# Autodesk Inventor assembly: placa
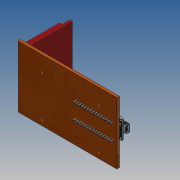
[picture p0: Inventor's stored thumbnail of the model, 180x180]
Saved by Autodesk Inventor 2017 (Build 210142000, 142)
## iProperties
Part Number: placa
Material: Genérico
Document SubType Name: Assembly
Designer: Leo
Author: Leo
## Documents named in this file (5)
- C:\Users\leo.DESKTOP-592E5E6\Dropbox\multiactuador\placa.iam
- C:\Users\leo.DESKTOP-592E5E6\Dropbox\multiactuador\placa\placa circuito.ipt
- C:\Users\leo.DESKTOP-592E5E6\Dropbox\multiactuador\import\arduino nano.ipt
- C:\Users\leo.DESKTOP-592E5E6\Dropbox\multiactuador\componentes\pantalla.ipt
- C:\Users\leo.DESKTOP-592E5E6\Dropbox\multiactuador\componentes\conector mini usb.ipt
## Components (4 placed, 4 different names)
1. placa circuito:1 — Nivelación:1, Coincidencia:1, Coincidencia:2, Nivelación:2, Coincidencia:3, Flush:4
2. arduino nano:1 — Nivelación:1, Coincidencia:1, Flush:5
3. pantalla:1 — Nivelación:2, Nivelación:3, Coincidencia:3
4. conector mini usb:1 — Coincidencia:2, Flush:4
## Relationships (8: Flush 5, Mate 3)
- Nivelación:1 [Flush]: placa circuito:1 ↔ arduino nano:1
- Coincidencia:1 [Mate]: placa circuito:1 ↔ arduino nano:1
- Coincidencia:2 [Mate] (3 mm): placa circuito:1 ↔ conector mini usb:1
- Nivelación:2 [Flush]: placa circuito:1 ↔ pantalla:1
- Nivelación:3 [Flush]: pantalla:1
- Coincidencia:3 [Mate] (3 mm): placa circuito:1 ↔ pantalla:1
- Flush:4 (12 mm): placa circuito:1 ↔ conector mini usb:1
- Flush:5 (-8 mm): arduino nano:1
